# Autodesk Inventor assembly: Button Fixture Assembly
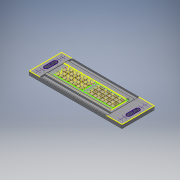
[picture p0: Inventor's stored thumbnail of the model, 180x180]
Saved by Autodesk Inventor 2016 (Build 200138000, 138)
## iProperties
Created: 2016-07-07
Part Number: Button Fixture Assembly
Document SubType Name: Assembly
Designer: Sam Clay
Author: Sam Clay
## Documents named in this file (3)
- Z:\enclosure\inventor\Button Fixture Assembly.iam
- Z:\enclosure\inventor\Button Fixture Base.ipt
- Z:\enclosure\inventor\Case Buttons CAM.ipt
## Components (17 placed, 2 different names)
1. Button Fixture Base:1 — Planar:2, Mate:1, Mate:2, Planar:3
2. Case Buttons CAM:9 — Planar:3
3. Case Buttons CAM:10
4. Case Buttons CAM:11
5. Case Buttons CAM:12
6. Case Buttons CAM:13
7. Case Buttons CAM:14
8. Case Buttons CAM:15
9. Case Buttons CAM:16
10. Case Buttons CAM:1 — Planar:2, Mate:1, Mate:2
11. Case Buttons CAM:2
12. Case Buttons CAM:3
13. Case Buttons CAM:4
14. Case Buttons CAM:5
15. Case Buttons CAM:6
16. Case Buttons CAM:7
17. Case Buttons CAM:8
## Component patterns: (1 elements), (8 elements, first: Case Buttons CAM:9), (8 elements, first: Case Buttons CAM:1)
## Relationships (4: PlanarJoint 2, Mate 2)
- Planar:2: Button Fixture Base:1 ↔ Case Buttons CAM:1
- Mate:1 (3.175 mm): Button Fixture Base:1 ↔ Case Buttons CAM:1
- Mate:2 (6.35 mm): Button Fixture Base:1 ↔ Case Buttons CAM:1
- Planar:3: Button Fixture Base:1 ↔ Case Buttons CAM:9
